# Autodesk Inventor assembly: centering
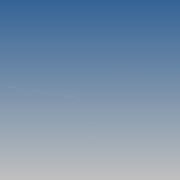
[picture p0: Inventor's stored thumbnail of the model, 180x180]
Saved by Autodesk Inventor 2014 SP1 (Build 180222100, 222)
## iProperties
Created: 2014-08-29
Part Number: centering
Document SubType Name: Assembly
Designer: Dave
Author: Dave
## Documents named in this file (4)
- C:\Users\Dave\Desktop\hera-cad\jigs\centering.iam
- C:\Users\Dave\Desktop\hera-cad\jigs\centeringKevlar.ipt
- C:\Users\Dave\Desktop\hera-cad\smallParts\spring.ipt
- C:\Users\Dave\Desktop\hera-cad\jigs\centeringRing.ipt
## Components (7 placed, 3 different names)
1. centeringRing:1 — Insert:2
2. centeringKevlar:1 — Insert:1, Insert:2
3. spring:1 — Insert:1
4. centeringKevlar:2
5. spring:2
6. centeringKevlar:3
7. spring:3
## Component patterns: (3 elements, first: centeringKevlar:1 + spring:1)
## Relationships (2: Insert 2)
- Insert:1: centeringKevlar:1 ↔ spring:1
- Insert:2: centeringRing:1 ↔ centeringKevlar:1
